# Autodesk Inventor assembly: legspacer
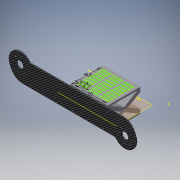
[picture p0: Inventor's stored thumbnail of the model, 180x180]
Saved by Autodesk Inventor 2018 (Build 220112000, 112)
## iProperties
Created: 2019-12-11
Part Number: legspacer
Document SubType Name: Assembly
Designer: bitbots
Author: bitbots
## Documents named in this file (3)
- C:\Users\bitbots\Desktop\bitbots_hardware\wolfgang\legspacer.iam
- C:\Users\bitbots\Desktop\bitbots_hardware\Part4.ipt
- C:\Users\bitbots\Desktop\bitbots_hardware\wolfgang\assembly\legs\lower_leg.ipt
## Components (2 placed, 2 different names)
1. lower_leg:1 — Mate:1, Angle:1, Flush:1
2. Part4:1 — Mate:1, Angle:1, Flush:1, Flush:2
## Relationships (4: Flush 2, Mate 1, Angle 1)
- Mate:1: lower_leg:1 ↔ Part4:1
- Angle:1 (0 deg): lower_leg:1 ↔ Part4:1
- Flush:1 (-2 mm): lower_leg:1 ↔ Part4:1
- Flush:2 (-19 mm): Part4:1
